# Autodesk Inventor assembly: Motor-Soporte-Montaje
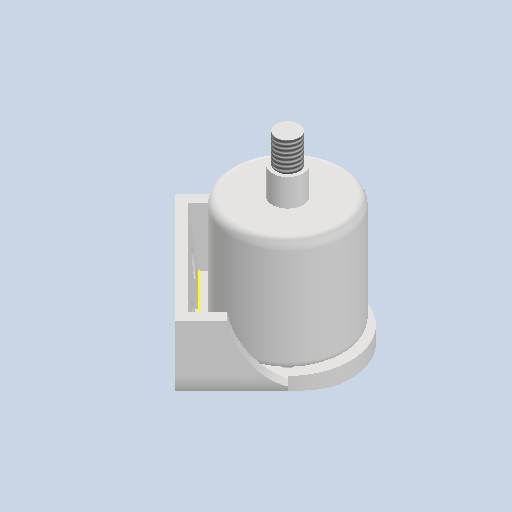
[picture p0: Inventor's stored thumbnail of the model, 512x512]
Saved by Autodesk Inventor 2024 (Build 280153000, 153)
## iProperties
Created: 2023-11-20
Part Number: Motor-Soporte-Montaje
Document SubType Name: Assembly
Designer: felip
Author: felip
## Documents named in this file (3)
- C:\Users\felip\Downloads\Gemelo Digital V2\Motor-Soporte-Montaje.iam
- C:\Users\felip\Downloads\Gemelo Digital V2\SoporteV5.ipt
- C:\Users\felip\Downloads\Gemelo Digital V2\bldc MOTOR.ipt
## Components (2 placed, 2 different names)
1. SoporteV5:1 — Rotational:1
2. bldc MOTOR:1 — Rotational:1
## Relationships (1: RevoluteJoint 1)
- Rotational:1 [RevoluteJoint]: SoporteV5:1 ↔ bldc MOTOR:1
